# Autodesk Inventor assembly: Assembly1
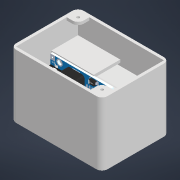
[picture p0: Inventor's stored thumbnail of the model, 180x180]
Saved by Autodesk Inventor 2022 (Build 260153000, 153)
## iProperties
Created: 2022-06-22
Part Number: Assembly1
Document SubType Name: Assembly
Designer: Gugarauj07
Author: Gugarauj07
## Documents named in this file (4)
- C:\Users\Gugarauj07\PycharmProjects\Eletronica_2022\CADS\Bike_Telemetry\Assembly1.iam
- C:\Users\Gugarauj07\PycharmProjects\Eletronica_2022\CADS\Bike_Telemetry\Bike_Telemetry.ipt
- C:\Users\Gugarauj07\PycharmProjects\Eletronica_2022\CADS\Bike_Telemetry\9v Duracell Body-Plain.ipt
- C:\Users\Gugarauj07\PycharmProjects\Eletronica_2022\CADS\Bike_Telemetry\LM2596 DC to DC Buck Converter 3 A.iam
## Components (3 placed, 3 different names)
1. Bike_Telemetry:1 — Mate:1, Mate:2
2. 9v Duracell Body-Plain:1 — Mate:1
3. LM2596 DC to DC Buck Converter 3 A:1 [sub-assembly] — Mate:2
## Relationships (2: Mate 2)
- Mate:1: Bike_Telemetry:1 ↔ 9v Duracell Body-Plain:1
- Mate:2 (-0.508 mm): Bike_Telemetry:1 ↔ LM2596 DC to DC Buck Converter 3 A:1
